# Autodesk Inventor assembly: BackMountAssembly_SimplfiedVersion
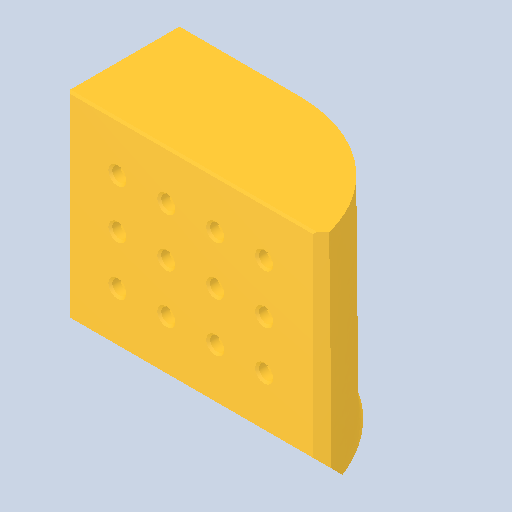
[picture p0: Inventor's stored thumbnail of the model, 512x512]
Saved by Autodesk Inventor 2022 (Build 260153000, 153)
## iProperties
Created: 2019-05-05
Part Number: BackMountAssembly_SimplfiedVersion
Document SubType Name: Assembly
Designer: lgnds
Author: lgnds
## Documents named in this file (2)
- C:\Users\lgnds\Documents\GitHub\MARV-Hardware-Mechanical\InventorProjects\FMS - Front Mounting System\FästenFörRam\BackMountAssembly_SimplfiedVersion.iam
- C:\Users\lgnds\Documents\GitHub\MARV-Hardware-Mechanical\InventorProjects\FMS - Front Mounting System\FästenFörRam\BakV4_SimplifiedVersionV2.ipt
## Components (1 placed, 1 different names)
1. BakV4_SimplifiedVersionV2:1 — Mate:1, Flush:1, Flush:2
## Relationships (3: Flush 2, Mate 1)
- Mate:1 (183 mm): BakV4_SimplifiedVersionV2:1
- Flush:1 (58 mm): BakV4_SimplifiedVersionV2:1
- Flush:2 (-45 mm): BakV4_SimplifiedVersionV2:1
